# Autodesk Inventor assembly: IntakeSlides3.0
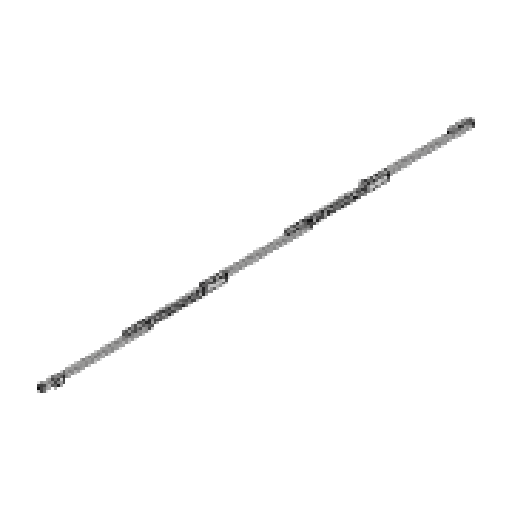
[picture p0: Inventor's stored thumbnail of the model, 512x512]
Saved by Autodesk Inventor 2023 (Build 270158000, 158)
## iProperties
Created: 2022-09-16
Part Number: IntakeSlides3.0
Document SubType Name: Assembly
Designer: deli
Author: deli
## Documents named in this file (5)
- C:\Users\deli\OneDrive - Eastside Preparatory School\FTC\8103-power-play\CAD\IntakeSlides3.0.iam
- C:\Users\deli\OneDrive - Eastside Preparatory School\FTC\8103-power-play\CAD\SlideStopBearingHolder.ipt
- C:\Users\deli\OneDrive - Eastside Preparatory School\FTC\8103-power-play\CAD\Rail.ipt
- C:\Users\deli\OneDrive - Eastside Preparatory School\FTC\8103-power-play\CAD\Carrige.ipt
- C:\Users\deli\OneDrive - Eastside Preparatory School\FTC\8103-power-play\CAD\Connector Plate.ipt
## Components (25 placed, 4 different names)
1. Carrige:1 — Mate:1, Flush:1, Flush:2, Mate:2, Mate:3, Flush:3
2. Carrige:2 — Mate:1, Flush:1, Flush:2
3. Rail:1 — Mate:2, Mate:3, Flush:3, Mate:5, Flush:6, Flush:7, Mate:34, Mate:35, Mate:43, Mate:50
4. Carrige:3 — Mate:6, Flush:8
5. Carrige:4 — Mate:7, Mate:8, Mate:9, Mate:10
6. Rail:2 — Mate:5, Flush:6, Flush:7, Mate:6, Mate:7, Flush:8, Mate:36, Mate:51
7. Connector Plate:1 — Mate:8, Mate:9, Mate:10, Mate:21, Mate:22, Mate:23
8. Carrige:5
9. Carrige:6 — Mate:21, Mate:22, Mate:23
10. Rail:3 — Mate:37, Mate:38, Mate:44, Mate:48
11. Carrige:7
12. Carrige:8
13. Rail:4 — Mate:39, Mate:49
14. Connector Plate:2 — Mate:31, Mate:32, Mate:33
15. Carrige:9
16. Carrige:10 — Mate:31, Mate:32, Mate:33
17. Rail:5 — Mate:40, Mate:41, Mate:45, Mate:46
18. Rail:6 — Mate:42, Mate:47, Mate:52, Mate:53
19. SlideStopBearingHolder:1 — Mate:43, Mate:50, Mate:51
20. SlideStopBearingHolder:2 — Mate:44, Mate:48, Mate:49
21. SlideStopBearingHolder:3 — Mate:45, Mate:46, Mate:47, Mate:54
22. SlideStopBearingHolder:4 — Mate:37, Mate:38, Mate:39
23. SlideStopBearingHolder:5 — Mate:40, Mate:41, Mate:42
24. SlideStopBearingHolder:6 — Mate:34, Mate:35, Mate:36
25. Carrige:11 — Mate:52, Mate:53, Mate:54
## Relationships (72: Mate 51, Flush 21)
- Mate:1: Carrige:1 ↔ Carrige:2
- Flush:1: Carrige:1 ↔ Carrige:2
- Flush:2: Carrige:1 ↔ Carrige:2
- Mate:2: Carrige:1 ↔ Rail:1
- Mate:3: Carrige:1 ↔ Rail:1
- Flush:3: Carrige:1 ↔ Rail:1
- [Mate]: Carrige:3 ↔ Carrige:4
- [Flush]: Carrige:3 ↔ Carrige:4
- [Flush]: Carrige:3 ↔ Carrige:4
- Mate:5: Rail:1 ↔ Rail:2
- Flush:6: Rail:1 ↔ Rail:2
- Flush:7: Rail:1 ↔ Rail:2
- Mate:6: Carrige:3 ↔ Rail:2
- Mate:7: Carrige:4 ↔ Rail:2
- Flush:8: Carrige:3 ↔ Rail:2
- Mate:8: Carrige:4 ↔ Connector Plate:1
- Mate:9: Carrige:4 ↔ Connector Plate:1
- Mate:10: Carrige:4 ↔ Connector Plate:1
- [Mate]: Carrige:5 ↔ Carrige:6
- [Flush]: Carrige:5 ↔ Carrige:6
- [Flush]: Carrige:5 ↔ Carrige:6
- [Mate]: Carrige:5 ↔ Rail:3
- [Mate]: Carrige:5 ↔ Rail:3
- [Flush]: Carrige:5 ↔ Rail:3
- [Mate]: Carrige:7 ↔ Carrige:8
- [Flush]: Carrige:7 ↔ Carrige:8
- [Flush]: Carrige:7 ↔ Carrige:8
- [Mate]: Rail:3 ↔ Rail:4
- [Flush]: Rail:3 ↔ Rail:4
- [Flush]: Rail:3 ↔ Rail:4
- [Mate]: Carrige:7 ↔ Rail:4
- [Mate]: Carrige:8 ↔ Rail:4
- [Flush]: Carrige:7 ↔ Rail:4
- [Mate]: Carrige:8 ↔ Connector Plate:2
- [Mate]: Carrige:8 ↔ Connector Plate:2
- [Mate]: Carrige:8 ↔ Connector Plate:2
- Mate:21: Connector Plate:1 ↔ Carrige:6
- Mate:22: Connector Plate:1 ↔ Carrige:6
- Mate:23: Connector Plate:1 ↔ Carrige:6
- [Mate]: Carrige:9 ↔ Carrige:10
- [Flush]: Carrige:9 ↔ Carrige:10
- [Flush]: Carrige:9 ↔ Carrige:10
- [Mate]: Carrige:9 ↔ Rail:5
- [Mate]: Carrige:9 ↔ Rail:5
- [Flush]: Carrige:9 ↔ Rail:5
- [Mate]: Rail:5 ↔ Rail:6
- [Flush]: Rail:5 ↔ Rail:6
- [Flush]: Rail:5 ↔ Rail:6
- Mate:31: Connector Plate:2 ↔ Carrige:10
- Mate:32: Connector Plate:2 ↔ Carrige:10
- Mate:33: Connector Plate:2 ↔ Carrige:10
- Mate:34: Rail:1 ↔ SlideStopBearingHolder:6
- Mate:35: Rail:1 ↔ SlideStopBearingHolder:6
- Mate:36: Rail:2 ↔ SlideStopBearingHolder:6
- Mate:37: Rail:3 ↔ SlideStopBearingHolder:4
- Mate:38: Rail:3 ↔ SlideStopBearingHolder:4
- Mate:39: Rail:4 ↔ SlideStopBearingHolder:4
- Mate:40: Rail:5 ↔ SlideStopBearingHolder:5
- Mate:41: Rail:5 ↔ SlideStopBearingHolder:5
- Mate:42: Rail:6 ↔ SlideStopBearingHolder:5
- Mate:43: Rail:1 ↔ SlideStopBearingHolder:1
- Mate:44: Rail:3 ↔ SlideStopBearingHolder:2
- Mate:45: Rail:5 ↔ SlideStopBearingHolder:3
- Mate:46: Rail:5 ↔ SlideStopBearingHolder:3
- Mate:47: Rail:6 ↔ SlideStopBearingHolder:3
- Mate:48: Rail:3 ↔ SlideStopBearingHolder:2
- Mate:49: Rail:4 ↔ SlideStopBearingHolder:2
- Mate:50: Rail:1 ↔ SlideStopBearingHolder:1
- Mate:51: Rail:2 ↔ SlideStopBearingHolder:1
- Mate:52: Rail:6 ↔ Carrige:11
- Mate:53: Rail:6 ↔ Carrige:11
- Mate:54 (271.1 mm): SlideStopBearingHolder:3 ↔ Carrige:11
## Named parameters: stroke = 0 mm, d55_d50 = 0 mm, d56_d51 = 0 mm, d57_d49 = 0 mm, d67_d50 = 0 mm, d68_d51 = 0 mm, d69_d52 = 0 mm, d70_d53 = 0 mm, d71_d54 = 0 mm, d72_d55_d50 = 0 mm, d73_d56_d51 = 0 mm, d74_d57_d49 = 0 mm, d75_d58 = 0 mm, d76_d59 = 0 mm, d77_d60 = 0 mm, d78_d61 = 0 mm, d79_d62 = 0 mm, d80_d63 = 0 mm, d81_d64 = 0 mm, d82_d65 = 0 mm, d83_d66 = 0 mm, d85_d49 = 0 mm, d89_d67_d50 = 0 mm, d90_d68_d51 = 0 mm, d91_d69_d52 = 0 mm, d92_d70_d53 = 0 mm, d93_d71_d54 = 0 mm, d97_d75_d58 = 0 mm, d98_d76_d59 = 0 mm, d99_d77_d60 = 0 mm, d104_d85_d49 = 0 mm
